# Autodesk Inventor assembly: Sponor Gift 2016-17
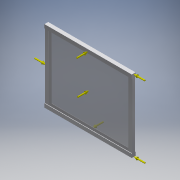
[picture p0: Inventor's stored thumbnail of the model, 180x180]
Saved by Autodesk Inventor 2016 (Build 200138000, 138)
## iProperties
Created: 2016-11-17
Part Number: Sponor Gift 2016-17
Document SubType Name: Assembly
Designer: 17kressc
Author: 17kressc
## Documents named in this file (12)
- C:\Users\17kressc\Documents\Sponor Gift 2016-17.iam
- C:\Users\17kressc\Documents\Large C Channel.ipt
- C:\Users\17kressc\Documents\Small C Channel.ipt
- C:\Users\17kressc\Documents\Plexi Sheet.ipt
- C:\Users\17kressc\Documents\Sponor Gift 2016-17\AIP\FEA\byuw6u8zk.fins
- C:\Users\17kressc\Documents\Sponor Gift 2016-17\AIP\FEA\byuw6u8zk.fsat
- C:\Users\17kressc\Documents\Sponor Gift 2016-17\AIP\FEA\byuw6u8zk.ftes
- C:\Users\17kressc\Documents\Sponor Gift 2016-17\AIP\FEA\byuw6u8zk.fwiz
- C:\Users\17kressc\Documents\Sponor Gift 2016-17\AIP\FEA\byuw6u934.fmsh
- C:\Users\17kressc\Documents\Sponor Gift 2016-17\AIP\FEA\byuw6u940.fres
- C:\Users\17kressc\Documents\Sponor Gift 2016-17\AIP\FEA\byuw6u98g.fmsh
- C:\Users\17kressc\Documents\Sponor Gift 2016-17\AIP\FEA\byuw6u98h.fres
## Components (6 placed, 3 different names)
1. Large C Channel:1 — Mate:1, Flush:1, Mate:2, Mate:3, Mate:4, Flush:2, Mate:8, Mate:11
2. Small C Channel:1 — Mate:1, Flush:1, Mate:2, Flush:3, Mate:5, Mate:6, Mate:12
3. Small C Channel:2 — Mate:3, Mate:4, Flush:2, Mate:7, Mate:9, Mate:13
4. Large C Channel:2 — Flush:3, Mate:5, Mate:6
5. Plexi Sheet:1 — Mate:7, Mate:8, Mate:9
6. Plexi Sheet:2 — Mate:11, Mate:12, Mate:13
## Relationships (15: Mate 12, Flush 3)
- Mate:1: Large C Channel:1 ↔ Small C Channel:1
- Flush:1: Large C Channel:1 ↔ Small C Channel:1
- Mate:2: Large C Channel:1 ↔ Small C Channel:1
- Mate:3: Large C Channel:1 ↔ Small C Channel:2
- Mate:4: Large C Channel:1 ↔ Small C Channel:2
- Flush:2: Large C Channel:1 ↔ Small C Channel:2
- Flush:3: Small C Channel:1 ↔ Large C Channel:2
- Mate:5: Small C Channel:1 ↔ Large C Channel:2
- Mate:6: Small C Channel:1 ↔ Large C Channel:2
- Mate:7: Small C Channel:2 ↔ Plexi Sheet:1
- Mate:8: Large C Channel:1 ↔ Plexi Sheet:1
- Mate:9: Small C Channel:2 ↔ Plexi Sheet:1
- Mate:11: Large C Channel:1 ↔ Plexi Sheet:2
- Mate:12: Small C Channel:1 ↔ Plexi Sheet:2
- Mate:13: Small C Channel:2 ↔ Plexi Sheet:2
## Named parameters: sa_0 = 0, sa_1 = -13344.7, sa_2 = 0, sa_3 = 0, sa_4 = 13344.7, sa_5 = 0, sa_6 = 444822, sa_7 = 0, sa_8 = 0, sa_9 = 2.22411e+06, sa_10 = 0, sa_11 = -1.03644e-10, sa_12 = -222411, sa_13 = 0, sa_14 = 0, sa_15 = -222411, sa_16 = 0, sa_17 = 5.20442e-11, sa_18 = 0, sa_19 = 0, sa_20 = -222411, sa_21 = 0, sa_22 = 0, sa_23 = -533787, sa_24 = 1.2455e-10, sa_25 = 0, sa_26 = 533787
note: some values were not read from the file. Shown as the stored number, unit unknown: "sa_0", "sa_1", "sa_2", "sa_3", "sa_4", "sa_5", "sa_6", "sa_7", "sa_8", "sa_9", "sa_10", "sa_11", "sa_12", "sa_13", "sa_14", "sa_15", "sa_16", "sa_17", "sa_18", "sa_19", "sa_20", "sa_21", "sa_22", "sa_23", "sa_24", "sa_25", "sa_26".
